# Autodesk Inventor assembly: Full-Assembly1
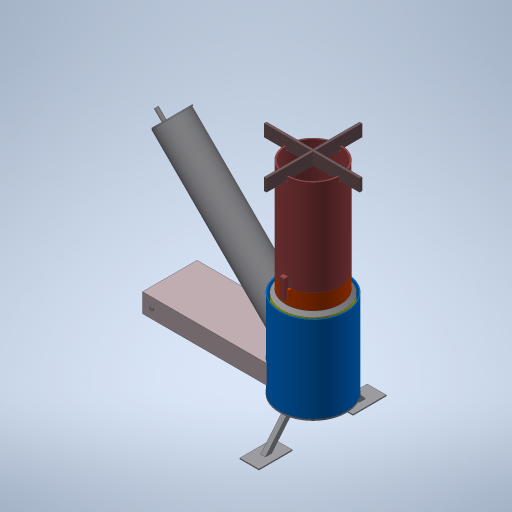
[picture p0: Inventor's stored thumbnail of the model, 512x512]
Saved by Autodesk Inventor 2024.3 (Build 283343000, 343)
## iProperties
Created: 2025-03-01
Part Number: Full-Assembly1
Document SubType Name: Assembly
Designer: ajclo
Author: ajclo
## Documents named in this file (11)
- C:\Users\ajclo\OneDrive - Stellenbosch University\Documents\BEng\Year IV\Skripsie\CAD\CAD Prototype 1\Full-Assembly1.iam
- C:\Users\ajclo\OneDrive - Stellenbosch University\Documents\BEng\Year IV\Skripsie\CAD\CAD Prototype 1\VerticalShaft.ipt
- C:\Users\ajclo\OneDrive - Stellenbosch University\Documents\BEng\Year IV\Skripsie\CAD\CAD Prototype 1\Insulation Shaft.ipt
- C:\Users\ajclo\OneDrive - Stellenbosch University\Documents\BEng\Year IV\Skripsie\CAD\CAD Prototype 1\Outer shaft.ipt
- C:\Users\ajclo\OneDrive - Stellenbosch University\Documents\BEng\Year IV\Skripsie\CAD\CAD Prototype 1\Slant.ipt
- C:\Users\ajclo\OneDrive - Stellenbosch University\Documents\BEng\Year IV\Skripsie\CAD\CAD Prototype 1\Cook-Assembly.iam
- C:\Users\ajclo\OneDrive - Stellenbosch University\Documents\BEng\Year IV\Skripsie\CAD\CAD Prototype 1\AirIntake.ipt
- C:\Users\ajclo\OneDrive - Stellenbosch University\Documents\BEng\Year IV\Skripsie\CAD\CAD Prototype 1\Feul_Intake.ipt
- C:\Users\ajclo\OneDrive - Stellenbosch University\Documents\BEng\Year IV\Skripsie\CAD\CAD Prototype 1\Bottom_plate.ipt
- C:\Users\ajclo\OneDrive - Stellenbosch University\Documents\BEng\Year IV\Skripsie\CAD\CAD Prototype 1\Air_Cotrol.ipt
- C:\Users\ajclo\OneDrive - Stellenbosch University\Documents\BEng\Year IV\Skripsie\CAD\CAD Prototype 1\Feul_ClosePlate.ipt
## Components (10 placed, 10 different names)
1. VerticalShaft:1 — Mate:1, Mate:2, Flush:1, Flush:2, Flush:4, Mate:5, Mate:6, Mate:7, Mate:8, Mate:9, Mate:10, Mate:11, Mate:13, Mate:20
2. Insulation Shaft:1 — Mate:2, Flush:1, Flush:3, Mate:12
3. Outer shaft:1 — Mate:1, Flush:2, Flush:3, Flush:4, Mate:21
4. Slant:1 — Mate:11, Mate:12
5. Cook-Assembly:1 [sub-assembly] — Mate:5, Mate:6, Mate:7, Flush:5
6. AirIntake:1 — Mate:8, Mate:9, Mate:10, Mate:16, Mate:17
7. Feul_Intake:1 — Mate:13, Flush:5, Mate:18, Mate:19
8. Bottom_plate:1 — Mate:20, Mate:21
9. Air_Cotrol:1 — Mate:16, Mate:17
10. Feul_ClosePlate:1 — Mate:18, Mate:19
## Relationships (22: Mate 17, Flush 5)
- Mate:1: VerticalShaft:1 ↔ Outer shaft:1
- Mate:2: VerticalShaft:1 ↔ Insulation Shaft:1
- Flush:1: VerticalShaft:1 ↔ Insulation Shaft:1
- Flush:2: VerticalShaft:1 ↔ Outer shaft:1
- Flush:3: Insulation Shaft:1 ↔ Outer shaft:1
- Flush:4: VerticalShaft:1 ↔ Outer shaft:1
- Mate:5: VerticalShaft:1 ↔ Cook-Assembly:1
- Mate:6: VerticalShaft:1 ↔ Cook-Assembly:1
- Mate:7 (1 mm): VerticalShaft:1 ↔ Cook-Assembly:1
- Mate:8: VerticalShaft:1 ↔ AirIntake:1
- Mate:9: VerticalShaft:1 ↔ AirIntake:1
- Mate:10: VerticalShaft:1 ↔ AirIntake:1
- Mate:11: VerticalShaft:1 ↔ Slant:1
- Mate:12: Insulation Shaft:1 ↔ Slant:1
- Mate:13: VerticalShaft:1 ↔ Feul_Intake:1
- Flush:5 (-40 mm): Cook-Assembly:1 ↔ Feul_Intake:1
- Mate:16: AirIntake:1 ↔ Air_Cotrol:1
- Mate:17: AirIntake:1 ↔ Air_Cotrol:1
- Mate:18: Feul_Intake:1 ↔ Feul_ClosePlate:1
- Mate:19: Feul_Intake:1 ↔ Feul_ClosePlate:1
- Mate:20: VerticalShaft:1 ↔ Bottom_plate:1
- Mate:21: Outer shaft:1 ↔ Bottom_plate:1
